# Autodesk Inventor assembly: NadelboxBaugruppe
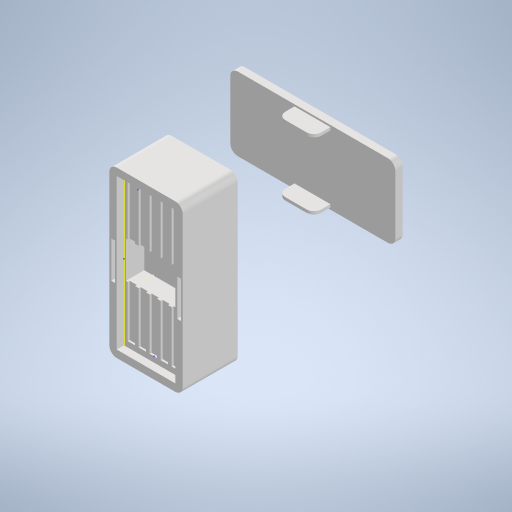
[picture p0: Inventor's stored thumbnail of the model, 512x512]
Saved by Autodesk Inventor 2023.1 (Build 271208000, 208)
## iProperties
Created: 2022-08-08
Part Number: NadelboxBaugruppe
Document SubType Name: Assembly
Designer: schwa
Author: schwa
## Documents named in this file (3)
- C:\3D_Drucker_Instruction_simplegcodeprints\NadelboxBaugruppe.iam
- C:\3D_Drucker_Instruction_simplegcodeprints\Nadelbox.ipt
- C:\3D_Drucker_Instruction_simplegcodeprints\NadelboxDeckel.ipt
## Components (2 placed, 2 different names)
1. Nadelbox:1 — Passend:1, Passend:2, Fluchtend:1, Passend:4, Passend:5, Passend:6, Fluchtend:2
2. NadelboxDeckel:1 — Passend:4, Passend:5, Passend:6, Fluchtend:2
## Relationships (7: Mate 5, Flush 2)
- Passend:1 [Mate]: Nadelbox:1
- Passend:2 [Mate]: Nadelbox:1
- Fluchtend:1 [Flush]: Nadelbox:1
- Passend:4 [Mate]: Nadelbox:1 ↔ NadelboxDeckel:1
- Passend:5 [Mate]: Nadelbox:1 ↔ NadelboxDeckel:1
- Passend:6 [Mate] (-6.5 mm): Nadelbox:1 ↔ NadelboxDeckel:1
- Fluchtend:2 [Flush]: Nadelbox:1 ↔ NadelboxDeckel:1
